# Autodesk Inventor assembly: battery holder
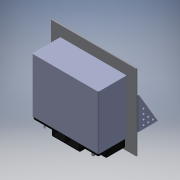
[picture p0: Inventor's stored thumbnail of the model, 180x180]
Saved by Autodesk Inventor 2016 (Build 200138000, 138)
## iProperties
Created: 2016-02-08
Part Number: battery holder
Document SubType Name: Assembly
Designer: gus
Mass: 2218.31 g
Surface Area: 1575.43 cm^2
Volume: 2218.31 cm^3
Density: 1 g/cm^3
Author: gus
## Documents named in this file (6)
- \\Mac\Home\Desktop\1510-stronghold-CAD-master\shooter\battery holder.iam
- \\Mac\Home\Desktop\1510-stronghold-CAD-master\shooter\plate.ipt
- \\Mac\Home\Desktop\1510-stronghold-CAD-master\batterystuff\User Library-Battery-6.ipt
- \\Mac\Home\Desktop\1510-stronghold-CAD-master\batterystuff\am-0477_Battery_Base.ipt
- \\Mac\Home\Desktop\1510-stronghold-CAD-master\batterystuff\am-3210L_Left_Bumper_Triangle_Bracket_AM14U3-2.ipt
- \\Mac\Home\Desktop\1510-stronghold-CAD-master\batterystuff\am-3210R_Right_Bumper_Triangle_Bracket_AM14U3-2.ipt
## Components (6 placed, 5 different names)
1. plate:1
2. User Library-Battery-6:1 — Mate:2, Flush:3, Mate:3
3. plate:2 — Mate:1, Mate:2, Flush:2, Flush:3, Mate:4, Mate:5, Flush:4, Mate:6, Flush:5, Flush:6, Flush:7
4. am-0477_Battery_Base:1 — Mate:1, Flush:2, Mate:3, Mate:4
5. am-3210L_Left_Bumper_Triangle_Bracket_AM14U3-2:1 — Mate:6, Flush:5, Flush:6
6. am-3210R_Right_Bumper_Triangle_Bracket_AM14U3-2:1 — Mate:5, Flush:4, Flush:7
## Relationships (12: Mate 6, Flush 6)
- Mate:1: plate:2 ↔ am-0477_Battery_Base:1
- Mate:2: User Library-Battery-6:1 ↔ plate:2
- Flush:2 (-67.945 mm): plate:2 ↔ am-0477_Battery_Base:1
- Flush:3 (25.4 mm): User Library-Battery-6:1 ↔ plate:2
- Mate:3: User Library-Battery-6:1 ↔ am-0477_Battery_Base:1
- Mate:4: plate:2 ↔ am-0477_Battery_Base:1
- Mate:5: plate:2 ↔ am-3210R_Right_Bumper_Triangle_Bracket_AM14U3-2:1
- Flush:4 (50.8 mm): plate:2 ↔ am-3210R_Right_Bumper_Triangle_Bracket_AM14U3-2:1
- Mate:6: plate:2 ↔ am-3210L_Left_Bumper_Triangle_Bracket_AM14U3-2:1
- Flush:5 (50.8 mm): plate:2 ↔ am-3210L_Left_Bumper_Triangle_Bracket_AM14U3-2:1
- Flush:6: plate:2 ↔ am-3210L_Left_Bumper_Triangle_Bracket_AM14U3-2:1
- Flush:7: plate:2 ↔ am-3210R_Right_Bumper_Triangle_Bracket_AM14U3-2:1
